# Autodesk Inventor assembly: planA
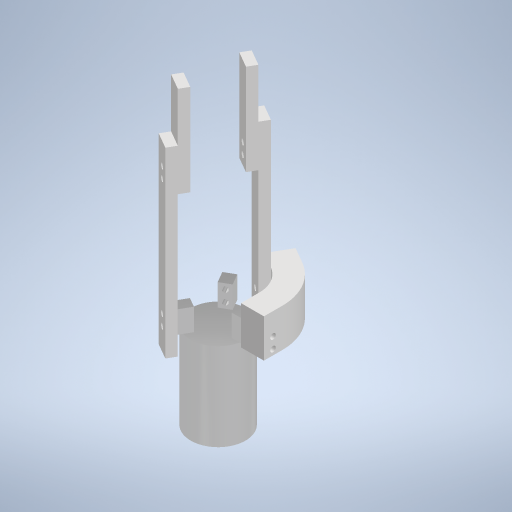
[picture p0: Inventor's stored thumbnail of the model, 512x512]
Saved by Autodesk Inventor 2024 (Build 280153000, 153)
## iProperties
Created: 2023-12-04
Part Number: planA
Document SubType Name: Assembly
Designer: Juan_Daleman
Author: Juan_Daleman
## Documents named in this file (5)
- D:\Documentos\Proyectos_U\Semestre 9\Robotica\Proyecto\PlanA\planA.iam
- D:\Documentos\Proyectos_U\Semestre 9\Robotica\Proyecto\PlanA\Cilindro.ipt
- D:\Documentos\Proyectos_U\Semestre 9\Robotica\Proyecto\PlanA\Soporte2_Dos.ipt
- D:\Documentos\Proyectos_U\Semestre 9\Robotica\Proyecto\PlanA\Soporte3_Dos.ipt
- D:\Documentos\Proyectos_U\Semestre 9\Robotica\Proyecto\PlanA\Soporte.ipt
## Components (6 placed, 4 different names)
1. Cilindro:1 — Insert:5, Insert:6, Insert:7, Insert:8
2. Soporte2_Dos:1 — Insert:1, Flush:1, Insert:9, Insert:10
3. Soporte2_Dos:2 — Flush:2, Insert:2, Insert:5, Insert:6
4. Soporte3_Dos:1 — Flush:2, Insert:2
5. Soporte3_Dos:2 — Insert:1, Flush:1
6. Soporte:1 — Insert:7, Insert:8, Insert:9, Insert:10
## Relationships (10: Insert 8, Flush 2)
- Insert:1: Soporte2_Dos:1 ↔ Soporte3_Dos:2
- Flush:1: Soporte2_Dos:1 ↔ Soporte3_Dos:2
- Flush:2: Soporte2_Dos:2 ↔ Soporte3_Dos:1
- Insert:2: Soporte2_Dos:2 ↔ Soporte3_Dos:1
- Insert:5: Cilindro:1 ↔ Soporte2_Dos:2
- Insert:6: Cilindro:1 ↔ Soporte2_Dos:2
- Insert:7: Cilindro:1 ↔ Soporte:1
- Insert:8: Cilindro:1 ↔ Soporte:1
- Insert:9: Soporte2_Dos:1 ↔ Soporte:1
- Insert:10: Soporte2_Dos:1 ↔ Soporte:1
